# Autodesk Inventor assembly: HbWristForChild
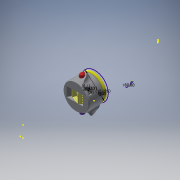
[picture p0: Inventor's stored thumbnail of the model, 180x180]
Saved by Autodesk Inventor 2017.3 (Build 213256000, 256)
## iProperties
Part Number: HbWristForChild
Material: 一般
Document SubType Name: Assembly
Designer: sktom
Author: sktom
## Documents named in this file (11)
- D:\CloudStrage\OneDrive\CAD\MAJ\hackberry\HACKberry-hardware\3D_69%\Inventor\HbWristForChild\HbWristForChild.iam
- D:\CloudStrage\OneDrive\CAD\MAJ\hackberry\HACKberry-hardware\3D_69%\Inventor\HbWristForChild\HBarmMountBase03ForChild.ipt
- D:\CloudStrage\OneDrive\CAD\MAJ\hackberry\HACKberry-hardware\3D_69%\Inventor\HbWristForChild\HBejectorLever02ForChild.ipt
- D:\CloudStrage\OneDrive\CAD\MAJ\hackberry\HACKberry-hardware\3D_69%\Inventor\HbWristForChild\HBabductionLever02forChild.ipt
- D:\CloudStrage\OneDrive\CAD\MAJ\hackberry\HACKberry-hardware\3D_69%\Inventor\HbWristForChild\CP 0.5-6-8.ipt
- D:\CloudStrage\OneDrive\CAD\MAJ\hackberry\HACKberry-hardware\3D_69%\Inventor\HbWristForChild\HBpronationLockPin02ForChild.ipt
- D:\CloudStrage\OneDrive\CAD\MAJ\hackberry\HACKberry-hardware\3D_69%\Inventor\HbWristForChild\HBlockPlateHolder02ForChild.ipt
- D:\CloudStrage\OneDrive\CAD\MAJ\hackberry\HACKberry-hardware\3D_69%\Inventor\HbWristForChild\HbWristLockPlate01ForChild.ipt
- D:\CloudStrage\OneDrive\CAD\MAJ\hackberry\HACKberry-hardware\3D_69%\Inventor\HbWristForChild\HBarmMount02ForChild.ipt
- D:\CloudStrage\OneDrive\CAD\MAJ\hackberry\HACKberry-hardware\3D_69%\Inventor\HbWristForChild\HBarmMountBaseCover03ForChild.ipt
- D:\CloudStrage\OneDrive\CAD\MAJ\hackberry\HACKberry-hardware\3D_69%\Inventor\HbWristForChild\SBI-SUJ-1d4.ipt
## Components (13 placed, 10 different names)
1. HBarmMountBase03ForChild:1 — 円柱状:1, メイト:1, 挿入:1, 挿入:2, 挿入:3, メイト:2, 挿入:4, 挿入:6, 挿入:10, 挿入:11
2. HBejectorLever02ForChild:1 — 円柱状:3, メイト:3
3. HBabductionLever02forChild:1 — 円柱状:1, メイト:1, 挿入:5
4. CP 0.5-6-8:1 — 挿入:1, 円柱状:2
5. CP 0.5-6-8:2 — 挿入:3
6. CP 0.5-6-8:3 — 挿入:2
7. HBpronationLockPin02ForChild:1 — 円柱状:2, メイト:2
8. HBlockPlateHolder02ForChild:1 — 挿入:4, 挿入:9
9. HBarmMount02ForChild:1 — 円柱状:3, 円柱状:4, メイト:3, 挿入:6
10. CP 0.5-6-8:4 — 挿入:5, 円柱状:4
11. HBarmMountBaseCover03ForChild:1 — 挿入:10, 挿入:11
12. SBI-SUJ-1d4:1
13. HbWristLockPlate01ForChild:1 — 挿入:9
## Relationships (16: Insert 9, CylindricalJoint 4, Mate 3)
- 円柱状:1 [CylindricalJoint]: HBarmMountBase03ForChild:1 ↔ HBabductionLever02forChild:1
- メイト:1 [Mate] (0.265 mm): HBarmMountBase03ForChild:1 ↔ HBabductionLever02forChild:1
- 挿入:1 [Insert]: HBarmMountBase03ForChild:1 ↔ CP 0.5-6-8:1
- 挿入:2 [Insert]: HBarmMountBase03ForChild:1 ↔ CP 0.5-6-8:3
- 挿入:3 [Insert]: HBarmMountBase03ForChild:1 ↔ CP 0.5-6-8:2
- 円柱状:2 [CylindricalJoint]: CP 0.5-6-8:1 ↔ HBpronationLockPin02ForChild:1
- メイト:2 [Mate] (0.265 mm): HBarmMountBase03ForChild:1 ↔ HBpronationLockPin02ForChild:1
- 挿入:4 [Insert]: HBarmMountBase03ForChild:1 ↔ HBlockPlateHolder02ForChild:1
- 円柱状:3 [CylindricalJoint]: HBejectorLever02ForChild:1 ↔ HBarmMount02ForChild:1
- 挿入:5 [Insert]: HBabductionLever02forChild:1 ↔ CP 0.5-6-8:4
- 円柱状:4 [CylindricalJoint]: HBarmMount02ForChild:1 ↔ CP 0.5-6-8:4
- メイト:3 [Mate] (0.3535 mm): HBejectorLever02ForChild:1 ↔ HBarmMount02ForChild:1
- 挿入:6 [Insert] (0.1 mm): HBarmMountBase03ForChild:1 ↔ HBarmMount02ForChild:1
- 挿入:9 [Insert]: HBlockPlateHolder02ForChild:1 ↔ HbWristLockPlate01ForChild:1
- 挿入:10 [Insert]: HBarmMountBase03ForChild:1 ↔ HBarmMountBaseCover03ForChild:1
- 挿入:11 [Insert]: HBarmMountBase03ForChild:1 ↔ HBarmMountBaseCover03ForChild:1
